# Autodesk Inventor assembly: 出幣機
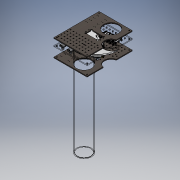
[picture p0: Inventor's stored thumbnail of the model, 180x180]
Saved by Autodesk Inventor 2017 (Build 210142000, 142)
## iProperties
Part Number: 出幣機
Material: 一般
Document SubType Name: Assembly
Designer: lygfy
Author: lygfy
## Documents named in this file (9)
- \\MissGAME-NAS\Miss GAME\松菸-幻影光靈\機關\出幣機\出幣機.iam
- \\MissGAME-NAS\Miss GAME\模型庫\MG995\MG995.ipt
- \\MissGAME-NAS\Miss GAME\松菸-幻影光靈\機關\出幣機\A0003.ipt
- \\MissGAME-NAS\Miss GAME\松菸-幻影光靈\機關\出幣機\A0001.ipt
- \\MissGAME-NAS\Miss GAME\松菸-幻影光靈\機關\出幣機\A0002.ipt
- \\MissGAME-NAS\Miss GAME\模型庫\HiLetgo ESP32\HiLetgo ESP32.iam
- \\MissGAME-NAS\Miss GAME\松菸-幻影光靈\機關\出幣機\A0004.ipt
- \\MissGAME-NAS\Miss GAME\模型庫\MG995\rychag_servo4.ipt
- \\MissGAME-NAS\Miss GAME\模型庫\A07-12.0\A07-12.0.iam
## Components (13 placed, 8 different names)
1. A0001:1 — 插入:1, 插入:2, 貼合:17, 貼合:18, 貼合:19, 貼合:21, 貼合:22, 貼合:24, 齊平:1, 齊平:2, 齊平:3, 齊平:4, 貼合:25
2. A0001:2 — 貼合:18, 貼合:19, 貼合:22, 插入:5, 插入:6
3. A0002:1 — 貼合:20, 插入:8, 貼合:23
4. A0003:1 — 貼合:17, 貼合:20
5. A0004:1 — 插入:5, 插入:6
6. A0001:3 — 齊平:3, 齊平:4, 貼合:25
7. HiLetgo ESP32:1 [sub-assembly] — 貼合:21
8. rychag_servo4:1 — 插入:7, 插入:8, 貼合:23
9. MG995:1 — 插入:1, 插入:2, 貼合:3, 貼合:4, 插入:7
10. A07-12.0:1 [sub-assembly] — 貼合:24, 齊平:1, 齊平:2
11. A07-12.0:2 [sub-assembly]
12. A07-12.0:3 [sub-assembly]
13. A07-12.0:4 [sub-assembly]
## Component patterns: (4 elements, first: A07-12.0:1)
## Relationships (21: Mate 11, Insert 6, Flush 4)
- 插入:1 [Insert]: A0001:1 ↔ MG995:1
- 插入:2 [Insert]: A0001:1 ↔ MG995:1
- 貼合:3 [Mate] (45 mm): MG995:1
- 貼合:4 [Mate]: MG995:1
- 貼合:17 [Mate]: A0001:1 ↔ A0003:1
- 貼合:18 [Mate]: A0001:1 ↔ A0001:2
- 貼合:19 [Mate]: A0001:1 ↔ A0001:2
- 貼合:20 [Mate] (1 mm): A0002:1 ↔ A0003:1
- 貼合:21 [Mate]: A0001:1 ↔ HiLetgo ESP32:1
- 貼合:22 [Mate] (20 mm): A0001:1 ↔ A0001:2
- 插入:5 [Insert]: A0001:2 ↔ A0004:1
- 插入:6 [Insert]: A0001:2 ↔ A0004:1
- 插入:7 [Insert]: rychag_servo4:1 ↔ MG995:1
- 插入:8 [Insert]: A0002:1 ↔ rychag_servo4:1
- 貼合:23 [Mate]: A0002:1 ↔ rychag_servo4:1
- 貼合:24 [Mate]: A0001:1 ↔ A07-12.0:1
- 齊平:1 [Flush] (4 mm): A0001:1 ↔ A07-12.0:1
- 齊平:2 [Flush] (14 mm): A0001:1 ↔ A07-12.0:1
- 齊平:3 [Flush]: A0001:1 ↔ A0001:3
- 齊平:4 [Flush]: A0001:1 ↔ A0001:3
- 貼合:25 [Mate] (30 mm): A0001:1 ↔ A0001:3
